# Autodesk Inventor assembly: Enclosure02
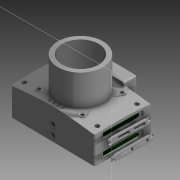
[picture p0: Inventor's stored thumbnail of the model, 180x180]
Saved by Autodesk Inventor 2013 (Build 170138000, 138)
## iProperties
Created: 2014-04-13
Part Number: Enclosure02
Document SubType Name: Assembly
Designer: spichelh
Author: spichelh
## Documents named in this file (17)
- C:\Users\spichelh\Documents\GitHub\beta-hardware\Enclosure\Version 002\Enclosure02.iam
- C:\Users\spichelh\Documents\GitHub\beta-hardware\Enclosure\Version 002\Enclosure01.ipt
- C:\Users\spichelh\Documents\GitHub\beta-hardware\Enclosure\Version 002\PCB01.ipt
- C:\Users\spichelh\Documents\GitHub\beta-hardware\Enclosure\Version 002\Microzed01.ipt
- C:\Users\spichelh\Documents\GitHub\beta-hardware\Enclosure\Version 002\AddonPCB01.ipt
- C:\Users\spichelh\Documents\GitHub\beta-hardware\Enclosure\Version 002\Enclosure-Backplate01.ipt
- C:\Users\spichelh\Documents\GitHub\beta-hardware\Enclosure\Version 002\Nikon Mount.ipt
- C:\Users\spichelh\Documents\GitHub\beta-hardware\Enclosure\Version 002\KAC12040.ipt
- C:\Users\spichelh\Documents\GitHub\beta-hardware\Enclosure\Version 002\IRGlass.ipt
- C:\Users\spichelh\Documents\GitHub\beta-hardware\Enclosure\Version 002\Cooler.ipt
- C:\Users\spichelh\Documents\GitHub\beta-hardware\Enclosure\Version 002\Enclosure02.ipt
- C:\Users\spichelh\Documents\GitHub\beta-hardware\Enclosure\Version 002\Nikon Mount 02.ipt
- C:\Users\spichelh\Documents\GitHub\beta-hardware\Enclosure\Version 002\Nikon Base 02.ipt
- C:\Users\spichelh\Documents\GitHub\beta-hardware\Enclosure\Version 002\IOModulePlate01.ipt
- C:\Users\spichelh\Documents\GitHub\beta-hardware\Enclosure\Version 002\PCBModule01.ipt
- C:\Users\spichelh\Documents\GitHub\beta-hardware\Enclosure\Version 002\PCBModuleLeft01.ipt
- C:\Users\spichelh\Documents\GitHub\beta-hardware\Enclosure\Version 002\IOModulePlate02.ipt
## Components (16 placed, 16 different names)
1. PCB01:1 — Mate:1, Flush:1, Flush:2, Mate:29, Flush:19, Flush:20, Mate:30, Flush:21, Flush:22, Flush:23, Insert:1
2. Microzed01:1 — Mate:1, Flush:1, Flush:2, Mate:2, Flush:22, Flush:24, Flush:25
3. AddonPCB01:1 — Mate:2, Flush:24, Flush:25
4. Nikon Mount:1 — Mate:20, Mate:21, Mate:22, Mate:26
5. Enclosure01:1 — Mate:26, Flush:16, Flush:17, Flush:18, Mate:27
6. Enclosure-Backplate01:1 — Flush:18, Mate:27
7. KAC12040:1
8. IRGlass:1 — Mate:20, Mate:21, Mate:22
9. Cooler:1 — Flush:16, Flush:17, Mate:35
10. Enclosure02:1 — Insert:2, Flush:26, Mate:33, Mate:34
11. Nikon Mount 02:1 — Mate:31, Mate:32, Insert:3
12. Nikon Base 02:1 — Mate:31, Mate:32, Insert:1, Flush:26, Mate:33, Mate:34, Insert:3, Mate:35
13. IOModulePlate01:1 — Insert:2
14. PCBModule01:1 — Mate:29, Flush:19, Flush:20
15. PCBModuleLeft01:1 — Mate:30, Flush:21, Flush:23
16. IOModulePlate02:1
## Relationships (30: Mate 14, Flush 13, Insert 3)
- Mate:1 (5 mm): PCB01:1 ↔ Microzed01:1
- Flush:1: PCB01:1 ↔ Microzed01:1
- Flush:2: PCB01:1 ↔ Microzed01:1
- Mate:2 (10 mm): Microzed01:1 ↔ AddonPCB01:1
- Mate:20: Nikon Mount:1 ↔ IRGlass:1
- Mate:21 (0.5 mm): Nikon Mount:1 ↔ IRGlass:1
- Mate:22 (0.5 mm): Nikon Mount:1 ↔ IRGlass:1
- Mate:26: Nikon Mount:1 ↔ Enclosure01:1
- Flush:16: Enclosure01:1 ↔ Cooler:1
- Flush:17 (33 mm): Enclosure01:1 ↔ Cooler:1
- Flush:18: Enclosure01:1 ↔ Enclosure-Backplate01:1
- Mate:27: Enclosure01:1 ↔ Enclosure-Backplate01:1
- Mate:29 (6 mm): PCB01:1 ↔ PCBModule01:1
- Flush:19: PCB01:1 ↔ PCBModule01:1
- Flush:20: PCB01:1 ↔ PCBModule01:1
- Mate:30 (6 mm): PCB01:1 ↔ PCBModuleLeft01:1
- Flush:21: PCB01:1 ↔ PCBModuleLeft01:1
- Flush:22: PCB01:1 ↔ Microzed01:1
- Flush:23: PCB01:1 ↔ PCBModuleLeft01:1
- Flush:24: Microzed01:1 ↔ AddonPCB01:1
- Flush:25: Microzed01:1 ↔ AddonPCB01:1
- Mate:31: Nikon Mount 02:1 ↔ Nikon Base 02:1
- Mate:32: Nikon Mount 02:1 ↔ Nikon Base 02:1
- Insert:1: PCB01:1 ↔ Nikon Base 02:1
- Insert:2 (10 mm): Enclosure02:1 ↔ IOModulePlate01:1
- Flush:26: Enclosure02:1 ↔ Nikon Base 02:1
- Mate:33: Enclosure02:1 ↔ Nikon Base 02:1
- Mate:34: Enclosure02:1 ↔ Nikon Base 02:1
- Insert:3: Nikon Mount 02:1 ↔ Nikon Base 02:1
- Mate:35: Cooler:1 ↔ Nikon Base 02:1
